# Autodesk Inventor assembly: uMule_board 1
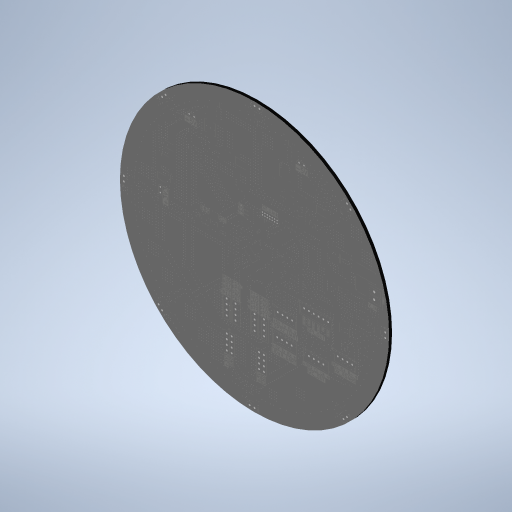
[picture p0: Inventor's stored thumbnail of the model, 512x512]
Saved by Autodesk Inventor 2024.3 (Build 283343000, 343)
## iProperties
Company: Kicad
Created: 2026-04-22
Part Number: uMule_board 1
Description: KiCad electronic assembly
Document SubType Name: Assembly
Designer: owozn
Authority: Unknown
Title: uMule_board.step
Author: Pcbnew
Sending System: KiCad to STEP converter
Preprocessor: Open CASCADE STEP processor 7.9
## Documents named in this file (6)
- C:\Users\owozn\Documents\Nauka\Studia\mgr\Semestr_3\Magisterka\temp\uMule\mechanics\subsets\uMule_board\uMule_board\uMule_board.iam
- C:\Users\owozn\Documents\Nauka\Studia\mgr\Semestr_3\Magisterka\temp\uMule\mechanics\subsets\uMule_board\uMule_board\uMule_board_silkscreen.ipt
- C:\Users\owozn\Documents\Nauka\Studia\mgr\Semestr_3\Magisterka\temp\uMule\mechanics\subsets\uMule_board\uMule_board\uMule_board_silkscreen_1.ipt
- C:\Users\owozn\Documents\Nauka\Studia\mgr\Semestr_3\Magisterka\temp\uMule\mechanics\subsets\uMule_board\uMule_board\uMule_board_soldermask.ipt
- C:\Users\owozn\Documents\Nauka\Studia\mgr\Semestr_3\Magisterka\temp\uMule\mechanics\subsets\uMule_board\uMule_board\uMule_board_soldermask_1.ipt
- C:\Users\owozn\Documents\Nauka\Studia\mgr\Semestr_3\Magisterka\temp\uMule\mechanics\subsets\uMule_board\uMule_board\uMule_board_PCB.ipt
## Components (5 placed, 5 different names)
1. 1
2. 2
3. 3
4. 4
5. 5
## Named parameters: Finish1_Area = 313.341
note: some values were not read from the file. Shown as the stored number, unit unknown: "Finish1_Area".
